# Autodesk Inventor assembly: 하단 조립품
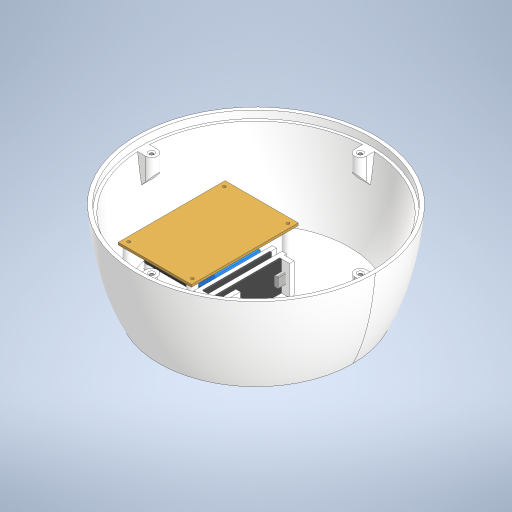
[picture p0: Inventor's stored thumbnail of the model, 512x512]
Saved by Autodesk Inventor 2023.1 (Build 271208000, 208)
## iProperties
Created: 2022-08-10
Part Number: 하단 조립품
Document SubType Name: Assembly
Designer: fly01
Author: fly01
## Documents named in this file (7)
- C:\Users\fly01\Desktop\PAI설계 2\조림품\하단 조립품.iam
- C:\Users\fly01\Desktop\PAI설계 2\출력품\body_bottom.ipt
- C:\Users\fly01\Desktop\PAI설계 2\조림품\하단 아크릴 조립품.iam
- C:\Users\fly01\Desktop\PAI설계 2\범용 부품\육각렌치볼트 m3 15mm.ipt
- C:\Users\fly01\Desktop\PAI설계 2\범용 부품\더블 릴레이 모듈.ipt
- C:\Users\fly01\Desktop\PAI설계 2\범용 부품\만능기판 소형.ipt
- C:\Users\fly01\Desktop\PAI설계 2\범용 부품\블루투스 모듈.ipt
## Components (10 placed, 6 different names)
1. body_bottom:1 — 삽입:1, 삽입:2, 삽입:4, 삽입:5, 삽입:6, 삽입:7, 메이트:1, 메이트:2, 메이트:3, 메이트:4
2. 하단 아크릴 조립품:1 [sub-assembly] — 삽입:1, 삽입:2, 삽입:3
3. 더블 릴레이 모듈:1 — 삽입:4, 삽입:5
4. 만능기판 소형:1 — 삽입:6, 삽입:7
5. 블루투스 모듈:1 — 메이트:1, 메이트:2
6. 블루투스 모듈:3 — 메이트:3, 메이트:4
7. 육각렌치볼트 m3 15mm:1 — 삽입:3
8. 육각렌치볼트 m3 15mm:2
9. 육각렌치볼트 m3 15mm:3
10. 육각렌치볼트 m3 15mm:4
## Component patterns: (4 elements, first: 육각렌치볼트 m3 15mm:1)
## Relationships (11: Insert 7, Mate 4)
- 삽입:1 [Insert] (-5 mm): body_bottom:1 ↔ 하단 아크릴 조립품:1
- 삽입:2 [Insert]: body_bottom:1 ↔ 하단 아크릴 조립품:1
- 삽입:3 [Insert]: 하단 아크릴 조립품:1 ↔ 육각렌치볼트 m3 15mm:1
- 삽입:4 [Insert]: body_bottom:1 ↔ 더블 릴레이 모듈:1
- 삽입:5 [Insert]: body_bottom:1 ↔ 더블 릴레이 모듈:1
- 삽입:6 [Insert]: body_bottom:1 ↔ 만능기판 소형:1
- 삽입:7 [Insert]: body_bottom:1 ↔ 만능기판 소형:1
- 메이트:1 [Mate]: body_bottom:1 ↔ 블루투스 모듈:1
- 메이트:2 [Mate]: body_bottom:1 ↔ 블루투스 모듈:1
- 메이트:3 [Mate]: body_bottom:1 ↔ 블루투스 모듈:3
- 메이트:4 [Mate]: body_bottom:1 ↔ 블루투스 모듈:3
